# Autodesk Inventor assembly: Assembly_Cube_Eyepiece_v3
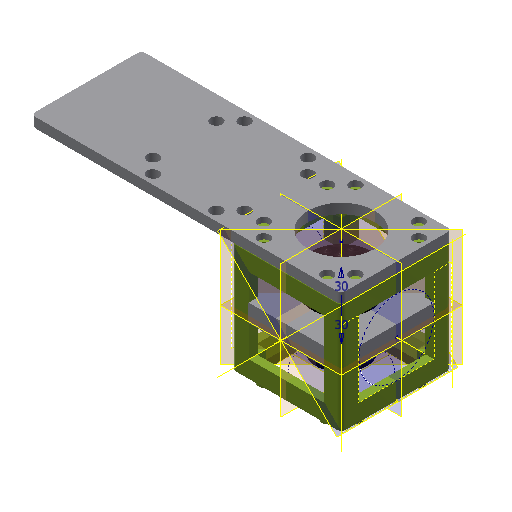
[picture p0: Inventor's stored thumbnail of the model, 512x512]
Saved by Autodesk Inventor 2022 (Build 260153000, 153)
## iProperties
Created: 2019-07-24
Part Number: Assembly_Cube_Eyepiece_v3
Document SubType Name: Assembly
Designer: marsikovabarbora
Author: marsikovabarbora
## Documents named in this file (5)
- C:\Users\PrakashLab\Documents\UC2-INVENTOR-Git\uc2_v3\Assembly_Cube_Eyepiece_v3.iam
- C:\Users\PrakashLab\Documents\UC2-INVENTOR-Git\uc2_v3\Assembly_Cube_empty_IM_v3.iam
- C:\Users\PrakashLab\Documents\UC2-INVENTOR-Git\uc2_v3\00_Eyepiece_WF20x 23,2mm.ipt
- C:\Users\PrakashLab\Documents\UC2-INVENTOR-Git\uc2_v3\30_Smartphone_Holder_v3.ipt
- C:\Users\PrakashLab\Documents\UC2-INVENTOR-Git\uc2_v3\20_Cube_Insert_Eyepiece.ipt
## Components (4 placed, 4 different names)
1. Assembly_Cube_empty_IM_v3:1 [sub-assembly] — Mate:3, Mate:4, Angle:1
2. 00_Eyepiece_WF20x 23,2mm:1 — Insert:1, Mate:9
3. 30_Smartphone_Holder_v3:1 — Mate:3, Mate:4, Angle:1, Mate:9
4. 20_Cube_Insert_Eyepiece:1 — Insert:1
## Relationships (9: Mate 7, Angle 1, Insert 1)
- Mate:3: Assembly_Cube_empty_IM_v3:1 ↔ 30_Smartphone_Holder_v3:1
- Mate:4: Assembly_Cube_empty_IM_v3:1 ↔ 30_Smartphone_Holder_v3:1
- Angle:1 (0 deg): Assembly_Cube_empty_IM_v3:1 ↔ 30_Smartphone_Holder_v3:1
- [Mate]: Assembly_Cube_empty_IM_v3:1 ↔ 20_Cube_Insert_Eyepiece:1
- [Mate]: 00_Eyepiece_WF20x 23,2mm:1 ↔ 20_Cube_Insert_Eyepiece:1
- [Mate]: 00_Eyepiece_WF20x 23,2mm:1 ↔ 20_Cube_Insert_Eyepiece:1
- [Mate]: Assembly_Cube_empty_IM_v3:1 ↔ 20_Cube_Insert_Eyepiece:1
- Insert:1: 00_Eyepiece_WF20x 23,2mm:1 ↔ 20_Cube_Insert_Eyepiece:1
- Mate:9: 00_Eyepiece_WF20x 23,2mm:1 ↔ 30_Smartphone_Holder_v3:1
